# Autodesk Inventor assembly: 組合(修改4-11)
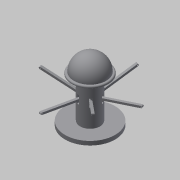
[picture p0: Inventor's stored thumbnail of the model, 180x180]
Saved by Autodesk Inventor 2018 (Build 220112000, 112)
## iProperties
Created: 2021-04-11
Part Number: 組合(修改4-11)
Material: 一般
Document SubType Name: Assembly
Designer: 王鼎鈞
Author: 王鼎鈞
## Documents named in this file (4)
- D:\2021顏家民\兩人組圖檔\組合(修改4-11).iam
- D:\2021顏家民\兩人組圖檔\支架4-9.ipt
- D:\2021顏家民\兩人組圖檔\主體4-9-1.ipt
- D:\2021顏家民\兩人組圖檔\凸輪設計4-9.ipt
## Components (8 placed, 3 different names)
1. 支架4-9:1 — 插入:3, 相切:3
2. 主體4-9-1:1 — 插入:3, 插入:4, 插入:5, 插入:6, 插入:7, 插入:8, 插入:9
3. 凸輪設計4-9:1 — 相切:1, 相切:2, 相切:3, 相切:4, 相切:5, 相切:6, 插入:9
4. 支架4-9:2 — 插入:4, 相切:2
5. 支架4-9:3 — 插入:5, 相切:1
6. 支架4-9:4 — 插入:6, 相切:5
7. 支架4-9:5 — 插入:7, 相切:4
8. 支架4-9:6 — 插入:8, 相切:6
## Relationships (13: Insert 7, Tangent 6)
- 插入:3 [Insert]: 支架4-9:1 ↔ 主體4-9-1:1
- 插入:4 [Insert]: 主體4-9-1:1 ↔ 支架4-9:2
- 插入:5 [Insert]: 主體4-9-1:1 ↔ 支架4-9:3
- 插入:6 [Insert]: 主體4-9-1:1 ↔ 支架4-9:4
- 插入:7 [Insert]: 主體4-9-1:1 ↔ 支架4-9:5
- 插入:8 [Insert]: 主體4-9-1:1 ↔ 支架4-9:6
- 相切:1 [Tangent]: 凸輪設計4-9:1 ↔ 支架4-9:3
- 相切:2 [Tangent]: 凸輪設計4-9:1 ↔ 支架4-9:2
- 相切:3 [Tangent]: 支架4-9:1 ↔ 凸輪設計4-9:1
- 相切:4 [Tangent]: 凸輪設計4-9:1 ↔ 支架4-9:5
- 相切:5 [Tangent]: 凸輪設計4-9:1 ↔ 支架4-9:4
- 相切:6 [Tangent]: 凸輪設計4-9:1 ↔ 支架4-9:6
- 插入:9 [Insert]: 主體4-9-1:1 ↔ 凸輪設計4-9:1
